# Autodesk Inventor assembly: IntakeExtensionBar_MIR1
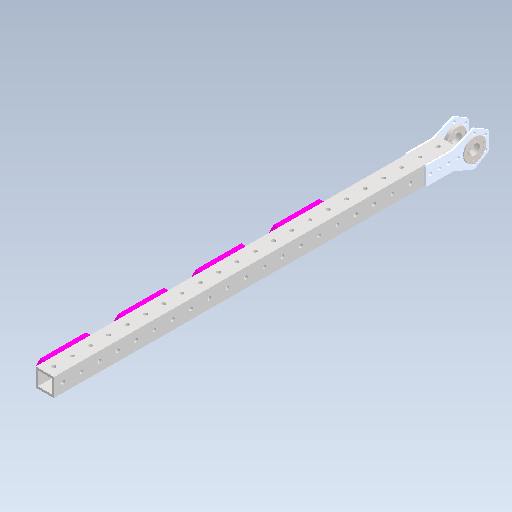
[picture p0: Inventor's stored thumbnail of the model, 512x512]
Saved by Autodesk Inventor 2020 (Build 240168000, 168)
## iProperties
Created: 2020-01-19
Part Number: IntakeExtensionBar_MIR1
Document SubType Name: Assembly
Designer: srini
Author: srini
## Documents named in this file (5)
- C:\Users\srini\Documents\FRC\2020\IntakeShooter\IntakeExtensionBar_MIR1.iam
- C:\Users\srini\Documents\FRC\2020\IntakeShooter\1x1x18_MIR1.ipt
- C:\Users\srini\Documents\FRC\2020\IntakeShooter\VersaFrame_End_Bearing_Gusset_217-3554_MIR1.ipt
- C:\Users\srini\Documents\FRC\2020\IntakeShooter\13_75mm_1_2_ThunderHex_ID_x_1_125_OD_x_0_313_WD_Flanged_Bearing_217-4006_MIR1.ipt
- C:\Users\srini\Documents\FRC\2020\IntakeShooter\ShaftRest_MIR1.ipt
## Components (9 placed, 4 different names)
1. 1x1x18_MIR1:1 — Insert:17, Insert:16, Insert:19, Insert:18, Insert:11, Insert:8, Insert:7, Insert:12, Insert:9, Insert:13, Insert:10, Insert:15, Insert:14
2. VersaFrame_End_Bearing_Gusset_217-3554_MIR1:1 — Insert:17, Insert:16, Insert:5
3. VersaFrame_End_Bearing_Gusset_217-3554_MIR1:2 — Insert:19, Insert:18, Insert:6
4. 13_75mm_1_2_ThunderHex_ID_x_1_125_OD_x_0_313_WD_Flanged_Bearing_217-4006_MIR1:1 — Insert:5
5. 13_75mm_1_2_ThunderHex_ID_x_1_125_OD_x_0_313_WD_Flanged_Bearing_217-4006_MIR1:2 — Insert:6
6. ShaftRest_MIR1:1 — Insert:11, Insert:8, Insert:7
7. ShaftRest_MIR1:2 — Insert:12, Insert:9
8. ShaftRest_MIR1:3 — Insert:13, Insert:10
9. ShaftRest_MIR1:4 — Insert:15, Insert:14
## Relationships (15: Insert 15)
- Insert:17: 1x1x18_MIR1:1 ↔ VersaFrame_End_Bearing_Gusset_217-3554_MIR1:1
- Insert:16: 1x1x18_MIR1:1 ↔ VersaFrame_End_Bearing_Gusset_217-3554_MIR1:1
- Insert:19: 1x1x18_MIR1:1 ↔ VersaFrame_End_Bearing_Gusset_217-3554_MIR1:2
- Insert:18: 1x1x18_MIR1:1 ↔ VersaFrame_End_Bearing_Gusset_217-3554_MIR1:2
- Insert:5: VersaFrame_End_Bearing_Gusset_217-3554_MIR1:1 ↔ 13_75mm_1_2_ThunderHex_ID_x_1_125_OD_x_0_313_WD_Flanged_Bearing_217-4006_MIR1:1
- Insert:6: VersaFrame_End_Bearing_Gusset_217-3554_MIR1:2 ↔ 13_75mm_1_2_ThunderHex_ID_x_1_125_OD_x_0_313_WD_Flanged_Bearing_217-4006_MIR1:2
- Insert:11: 1x1x18_MIR1:1 ↔ ShaftRest_MIR1:1
- Insert:8: 1x1x18_MIR1:1 ↔ ShaftRest_MIR1:1
- Insert:7: 1x1x18_MIR1:1 ↔ ShaftRest_MIR1:1
- Insert:12: 1x1x18_MIR1:1 ↔ ShaftRest_MIR1:2
- Insert:9: 1x1x18_MIR1:1 ↔ ShaftRest_MIR1:2
- Insert:13: 1x1x18_MIR1:1 ↔ ShaftRest_MIR1:3
- Insert:10: 1x1x18_MIR1:1 ↔ ShaftRest_MIR1:3
- Insert:15: 1x1x18_MIR1:1 ↔ ShaftRest_MIR1:4
- Insert:14: 1x1x18_MIR1:1 ↔ ShaftRest_MIR1:4
